# Autodesk Inventor assembly: Pivot Mount
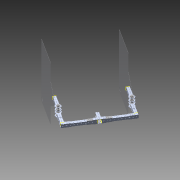
[picture p0: Inventor's stored thumbnail of the model, 180x180]
Saved by Autodesk Inventor 2014 (Build 180170000, 170)
## iProperties
Created: 2014-01-07
Part Number: Pivot Mount
Document SubType Name: Assembly
Designer: Michael
Mass: 1453.46 g
Surface Area: 4266.1 cm^2
Volume: 366.027 cm^3
Density: 3.97091 g/cm^3
Author: Michael
## Documents named in this file (11)
- C:\Users\Michael\Documents\GitHub\2014buildCAD\Funnel Catcher\Pivot Mount.iam
- C:\Users\Michael\Documents\GitHub\2014buildCAD\Funnel Catcher\Vex Pro End Bearing Mount.ipt
- C:\Users\Michael\Documents\GitHub\2014buildCAD\Funnel Catcher\Vex Pro 1x1 rectangular tubing 4 in length.ipt
- C:\Users\Michael\Documents\GitHub\2014buildCAD\Funnel Catcher\3-8 ID 1.125 OD Bearing (6384K348).ipt
- C:\Users\Michael\Documents\GitHub\2014buildCAD\Funnel Catcher\3-8 in ID shaft collar (6435K130).ipt
- C:\Users\Michael\Documents\GitHub\2014buildCAD\Funnel Catcher\Vex Pro T Gusset.ipt
- C:\Users\Michael\Documents\GitHub\2014buildCAD\Funnel Catcher\Vex Pro 1x1 rectangular tubing 7 in length.ipt
- C:\Users\Michael\Documents\GitHub\2014buildCAD\Funnel Catcher\4 in 3-8 diameter Shaft (6061K419).ipt
- C:\Users\Michael\Documents\GitHub\2014buildCAD\Funnel Catcher\Vex Pro 90 degree Gusset.ipt
- C:\Users\Michael\Documents\GitHub\2014buildCAD\Funnel Catcher\3 X 1 Spacer.ipt
- C:\Users\Michael\Documents\GitHub\2014buildCAD\Funnel Catcher\Funnel 2.ipt
## Components (44 placed, 10 different names)
1. Vex Pro End Bearing Mount:1
2. Vex Pro 1x1 rectangular tubing 4 in length:1 — Insert:113, Insert:114, Insert:118
3. Vex Pro End Bearing Mount:2
4. 3-8 ID 1.125 OD Bearing (6384K348):1 — Insert:70
5. 3-8 ID 1.125 OD Bearing (6384K348):2 — Insert:69
6. 3-8 in ID shaft collar (6435K130):1 — Insert:59
7. Vex Pro End Bearing Mount:3
8. Vex Pro 1x1 rectangular tubing 4 in length:2 — Insert:115, Insert:116, Insert:121, Angle:2
9. Vex Pro End Bearing Mount:4
10. 3-8 ID 1.125 OD Bearing (6384K348):3 — Insert:49
11. 3-8 ID 1.125 OD Bearing (6384K348):4 — Insert:50
12. 3-8 in ID shaft collar (6435K130):2 — Insert:50, Insert:55
13. Vex Pro End Bearing Mount:5 — Insert:57, Insert:58
14. Vex Pro End Bearing Mount:6 — Insert:51, Insert:52
15. 3-8 ID 1.125 OD Bearing (6384K348):5 — Insert:59
16. 3-8 ID 1.125 OD Bearing (6384K348):6 — Insert:55
17. 3-8 in ID shaft collar (6435K130):3 — Insert:48, Insert:49
18. Vex Pro 1x1 rectangular tubing 4 in length:4 — Insert:51, Insert:52, Insert:57, Insert:58, Insert:160, Insert:161, Angle:1, Angle:2
19. 4 in 3-8 diameter Shaft (6061K419):1 — Insert:66
20. 4 in 3-8 diameter Shaft (6061K419):2 — Insert:48
21. 3-8 in ID shaft collar (6435K130):5 — Insert:66, Insert:67
22. 3-8 in ID shaft collar (6435K130):6 — Insert:68, Insert:69
23. 3-8 in ID shaft collar (6435K130):8 — Insert:70
24. Vex Pro End Bearing Mount:7
25. Vex Pro End Bearing Mount:8
26. 3-8 ID 1.125 OD Bearing (6384K348):7 — Insert:67
27. 3-8 ID 1.125 OD Bearing (6384K348):8 — Insert:68
28. Vex Pro 1x1 rectangular tubing 4 in length:6 — Insert:158, Insert:159, Angle:1
29. Vex Pro 90 degree Gusset:1 — Insert:113, Insert:114, Insert:126, Insert:127
30. Vex Pro 90 degree Gusset:2 — Insert:115, Insert:116, Insert:129, Insert:130
31. Vex Pro 90 degree Gusset:3 — Insert:118, Insert:128
32. Vex Pro 90 degree Gusset:4 — Insert:121, Insert:131
33. Vex Pro 1x1 rectangular tubing 7 in length:3 — Insert:129, Insert:130, Insert:131, Insert:148, Insert:149, Insert:152, Insert:153
34. Vex Pro 1x1 rectangular tubing 7 in length:4 — Insert:126, Insert:127, Insert:128, Insert:150, Insert:151
35. 3 X 1 Spacer:1 — Insert:154, Insert:155
36. 3 X 1 Spacer:2 — Insert:156, Insert:157
37. Vex Pro T Gusset:1 — Insert:144, Insert:145, Insert:146, Insert:147, Insert:156, Insert:157
38. Vex Pro T Gusset:2 — Insert:138, Insert:139, Insert:140, Insert:141, Insert:154, Insert:155
39. 3 X 1 Spacer:3 — Insert:138, Insert:139, Insert:152, Insert:153
40. 3 X 1 Spacer:4 — Insert:146, Insert:147, Insert:148, Insert:149
41. 3 X 1 Spacer:5 — Insert:140, Insert:141
42. 3 X 1 Spacer:6 — Insert:144, Insert:145, Insert:150, Insert:151
43. Funnel 2:1 — Insert:158, Insert:159
44. Funnel 2:2 — Insert:160, Insert:161
## Relationships (70: Insert 68, Angle 2)
- [Insert]: Vex Pro End Bearing Mount:2 ↔ 3-8 ID 1.125 OD Bearing (6384K348):2
- [Insert]: Vex Pro End Bearing Mount:1 ↔ 3-8 ID 1.125 OD Bearing (6384K348):1
- [Insert]: Vex Pro End Bearing Mount:1 ↔ Vex Pro 1x1 rectangular tubing 4 in length:1
- [Insert]: Vex Pro 1x1 rectangular tubing 4 in length:1 ↔ Vex Pro End Bearing Mount:2
- [Insert]: Vex Pro End Bearing Mount:1 ↔ Vex Pro 1x1 rectangular tubing 4 in length:1
- [Insert]: Vex Pro 1x1 rectangular tubing 4 in length:1 ↔ Vex Pro End Bearing Mount:2
- [Insert]: Vex Pro End Bearing Mount:4 ↔ 3-8 ID 1.125 OD Bearing (6384K348):4
- [Insert]: Vex Pro End Bearing Mount:3 ↔ 3-8 ID 1.125 OD Bearing (6384K348):3
- [Insert]: Vex Pro End Bearing Mount:3 ↔ Vex Pro 1x1 rectangular tubing 4 in length:2
- [Insert]: Vex Pro 1x1 rectangular tubing 4 in length:2 ↔ Vex Pro End Bearing Mount:4
- [Insert]: Vex Pro End Bearing Mount:3 ↔ Vex Pro 1x1 rectangular tubing 4 in length:2
- [Insert]: Vex Pro 1x1 rectangular tubing 4 in length:2 ↔ Vex Pro End Bearing Mount:4
- [Insert]: Vex Pro End Bearing Mount:6 ↔ 3-8 ID 1.125 OD Bearing (6384K348):6
- [Insert]: Vex Pro End Bearing Mount:5 ↔ 3-8 ID 1.125 OD Bearing (6384K348):5
- Insert:48 (-1.27 mm): 3-8 in ID shaft collar (6435K130):3 ↔ 4 in 3-8 diameter Shaft (6061K419):2
- Insert:49: 3-8 ID 1.125 OD Bearing (6384K348):3 ↔ 3-8 in ID shaft collar (6435K130):3
- Insert:50: 3-8 ID 1.125 OD Bearing (6384K348):4 ↔ 3-8 in ID shaft collar (6435K130):2
- Insert:51: Vex Pro End Bearing Mount:6 ↔ Vex Pro 1x1 rectangular tubing 4 in length:4
- Insert:52: Vex Pro End Bearing Mount:6 ↔ Vex Pro 1x1 rectangular tubing 4 in length:4
- Insert:55: 3-8 in ID shaft collar (6435K130):2 ↔ 3-8 ID 1.125 OD Bearing (6384K348):6
- Insert:57: Vex Pro End Bearing Mount:5 ↔ Vex Pro 1x1 rectangular tubing 4 in length:4
- Insert:58: Vex Pro End Bearing Mount:5 ↔ Vex Pro 1x1 rectangular tubing 4 in length:4
- Insert:59: 3-8 in ID shaft collar (6435K130):1 ↔ 3-8 ID 1.125 OD Bearing (6384K348):5
- [Insert]: Vex Pro End Bearing Mount:8 ↔ 3-8 ID 1.125 OD Bearing (6384K348):8
- [Insert]: Vex Pro End Bearing Mount:7 ↔ 3-8 ID 1.125 OD Bearing (6384K348):7
- [Insert]: Vex Pro End Bearing Mount:8 ↔ Vex Pro 1x1 rectangular tubing 4 in length:6
- [Insert]: Vex Pro End Bearing Mount:8 ↔ Vex Pro 1x1 rectangular tubing 4 in length:6
- [Insert]: Vex Pro End Bearing Mount:7 ↔ Vex Pro 1x1 rectangular tubing 4 in length:6
- [Insert]: Vex Pro End Bearing Mount:7 ↔ Vex Pro 1x1 rectangular tubing 4 in length:6
- Insert:66: 4 in 3-8 diameter Shaft (6061K419):1 ↔ 3-8 in ID shaft collar (6435K130):5
- Insert:67: 3-8 in ID shaft collar (6435K130):5 ↔ 3-8 ID 1.125 OD Bearing (6384K348):7
- Insert:68: 3-8 in ID shaft collar (6435K130):6 ↔ 3-8 ID 1.125 OD Bearing (6384K348):8
- Insert:69: 3-8 ID 1.125 OD Bearing (6384K348):2 ↔ 3-8 in ID shaft collar (6435K130):6
- Insert:70: 3-8 ID 1.125 OD Bearing (6384K348):1 ↔ 3-8 in ID shaft collar (6435K130):8
- Insert:113: Vex Pro 1x1 rectangular tubing 4 in length:1 ↔ Vex Pro 90 degree Gusset:1
- Insert:114: Vex Pro 1x1 rectangular tubing 4 in length:1 ↔ Vex Pro 90 degree Gusset:1
- Insert:115: Vex Pro 1x1 rectangular tubing 4 in length:2 ↔ Vex Pro 90 degree Gusset:2
- Insert:116: Vex Pro 1x1 rectangular tubing 4 in length:2 ↔ Vex Pro 90 degree Gusset:2
- Insert:118: Vex Pro 1x1 rectangular tubing 4 in length:1 ↔ Vex Pro 90 degree Gusset:3
- Insert:121: Vex Pro 1x1 rectangular tubing 4 in length:2 ↔ Vex Pro 90 degree Gusset:4
- Insert:126: Vex Pro 90 degree Gusset:1 ↔ Vex Pro 1x1 rectangular tubing 7 in length:4
- Insert:127: Vex Pro 90 degree Gusset:1 ↔ Vex Pro 1x1 rectangular tubing 7 in length:4
- Insert:128: Vex Pro 90 degree Gusset:3 ↔ Vex Pro 1x1 rectangular tubing 7 in length:4
- Insert:129: Vex Pro 90 degree Gusset:2 ↔ Vex Pro 1x1 rectangular tubing 7 in length:3
- Insert:130: Vex Pro 90 degree Gusset:2 ↔ Vex Pro 1x1 rectangular tubing 7 in length:3
- Insert:131: Vex Pro 90 degree Gusset:4 ↔ Vex Pro 1x1 rectangular tubing 7 in length:3
- Insert:138: Vex Pro T Gusset:2 ↔ 3 X 1 Spacer:3
- Insert:139: Vex Pro T Gusset:2 ↔ 3 X 1 Spacer:3
- Insert:140: Vex Pro T Gusset:2 ↔ 3 X 1 Spacer:5
- Insert:141: Vex Pro T Gusset:2 ↔ 3 X 1 Spacer:5
- Insert:144: Vex Pro T Gusset:1 ↔ 3 X 1 Spacer:6
- Insert:145: Vex Pro T Gusset:1 ↔ 3 X 1 Spacer:6
- Insert:146: Vex Pro T Gusset:1 ↔ 3 X 1 Spacer:4
- Insert:147: Vex Pro T Gusset:1 ↔ 3 X 1 Spacer:4
- Insert:148: Vex Pro 1x1 rectangular tubing 7 in length:3 ↔ 3 X 1 Spacer:4
- Insert:149: Vex Pro 1x1 rectangular tubing 7 in length:3 ↔ 3 X 1 Spacer:4
- Insert:150: Vex Pro 1x1 rectangular tubing 7 in length:4 ↔ 3 X 1 Spacer:6
- Insert:151: Vex Pro 1x1 rectangular tubing 7 in length:4 ↔ 3 X 1 Spacer:6
- Insert:152: Vex Pro 1x1 rectangular tubing 7 in length:3 ↔ 3 X 1 Spacer:3
- Insert:153: Vex Pro 1x1 rectangular tubing 7 in length:3 ↔ 3 X 1 Spacer:3
- Insert:154: 3 X 1 Spacer:1 ↔ Vex Pro T Gusset:2
- Insert:155: 3 X 1 Spacer:1 ↔ Vex Pro T Gusset:2
- Insert:156: 3 X 1 Spacer:2 ↔ Vex Pro T Gusset:1
- Insert:157: 3 X 1 Spacer:2 ↔ Vex Pro T Gusset:1
- Insert:158: Vex Pro 1x1 rectangular tubing 4 in length:6 ↔ Funnel 2:1
- Insert:159: Vex Pro 1x1 rectangular tubing 4 in length:6 ↔ Funnel 2:1
- Insert:160: Vex Pro 1x1 rectangular tubing 4 in length:4 ↔ Funnel 2:2
- Insert:161: Vex Pro 1x1 rectangular tubing 4 in length:4 ↔ Funnel 2:2
- Angle:1 (0 deg): Vex Pro 1x1 rectangular tubing 4 in length:4 ↔ Vex Pro 1x1 rectangular tubing 4 in length:6
- Angle:2 (0 deg): Vex Pro 1x1 rectangular tubing 4 in length:2 ↔ Vex Pro 1x1 rectangular tubing 4 in length:4
## Named parameters: d3_d4 = 0 mm, d4_d5 = 0 mm, d8_d30 = 0 mm, d9_d31 = 0 mm, d10_d32 = 0 mm, d11_d3_d4 = 0 mm, d12_d4_d5 = 0 mm, d14_d25 = 0 mm, d18_d3_d4 = 0 mm, d19_d4_d5 = 0 mm, d66_d63 = 0 mm, d67_d64 = 0 mm, d68_d57 = 0 mm, d69_d58 = 0 mm, d70_d18_d3_d4 = 0 mm, d71_d19_d4_d5 = 0 mm
